# Autodesk Inventor assembly: kbd
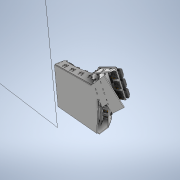
[picture p0: Inventor's stored thumbnail of the model, 180x180]
Saved by Autodesk Inventor 2020 (Build 240168000, 168)
## iProperties
Created: 2019-07-12
Part Number: kbd
Document SubType Name: Assembly
Designer: Thibault
Author: Thibault
## Documents named in this file (4)
- C:\Users\Thibault Polge\Documents\Habilis\mech\kbd.iam
- C:\Users\Thibault Polge\Documents\Habilis\mech\keywell.iam
- C:\Users\Thibault Polge\Documents\Habilis\mech\tc_switchplate.iam
- C:\Users\Thibault Polge\Documents\Habilis\mech\base_plate.ipt
## Components (3 placed, 3 different names)
1. keywell:1 [sub-assembly] — Affleurement:1, Placage:1, Affleurement:2, Affleurement:3
2. tc_switchplate:1 [sub-assembly] — Affleurement:1
3. base_plate:1 — Placage:1, Affleurement:2, Affleurement:3
## Relationships (4: Flush 3, Mate 1)
- Affleurement:1 [Flush]: keywell:1 ↔ tc_switchplate:1
- Placage:1 [Mate]: keywell:1 ↔ base_plate:1
- Affleurement:2 [Flush]: keywell:1 ↔ base_plate:1
- Affleurement:3 [Flush]: keywell:1 ↔ base_plate:1
